# Autodesk Inventor assembly: BG301_trajan20_21
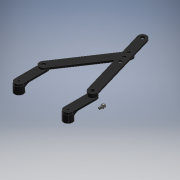
[picture p0: Inventor's stored thumbnail of the model, 180x180]
Saved by Autodesk Inventor 2022.2 (Build 262287000, 287)
## iProperties
Company: HTBLA Kaindorf
RuleStatus: InUse
Created: 2022-08-22
Part Number: BG301_trajan20_21
Project: Zeichenmaschine_v2
Material: Generisch
Description: gelenke
Document SubType Name: Assembly
Designer: trajan20
AfterDocNew0: iProperties-Editor_aufrufen
Author: jan
Keywords: 2021
## Documents named in this file (6)
- C:\Users\jan\Documents\DrawMachine\DrawMachineConstruction\Projekt\Zeichenmaschine_v2\BG301_trajan20_21_Zeichenmaschine_v2_gelenke.iam
- C:\Users\jan\Documents\DrawMachine\DrawMachineConstruction\Projekt\Zeichenmaschine_v2\BT301_trajan20_21_Zeichenmaschine_v2_gelenk 1.ipt
- C:\Users\jan\Documents\DrawMachine\DrawMachineConstruction\Projekt\Zeichenmaschine_v2\BT301_trajan20_21_Zeichenmaschine_v2_gelenk a.ipt
- C:\Users\jan\Documents\DrawMachine\DrawMachineConstruction\Projekt\Zeichenmaschine_v2\BT303_trajan20_21_Zeichenmaschine_v2_gelenk b.ipt
- C:\Users\jan\Documents\DrawMachine\DrawMachineConstruction\Projekt\Zeichenmaschine_v2\BT305_trajan20_21_Zeichenmaschine_v2_Platzhalter_steppermotor.ipt
- C:\Users\jan\Documents\DrawMachine\DrawMachineConstruction\Projekt\Zeichenmaschine_v2\Normteile\de-DE\ISO 4762(2)\ISO 4762 - M5 x 8ISO.ipt
## Components (7 placed, 5 different names)
1. BT301_trajan20_21_Zeichenmaschine_v2_gelenk 1:1 — Passend:1, Fluchtend:1, Winkel:1, Passend:9, Passend:15, Passend:16
2. BT301_trajan20_21_Zeichenmaschine_v2_gelenk a:1 — Passend:2, Passend:3, Passend:18
3. BT301_trajan20_21_Zeichenmaschine_v2_gelenk 1:2 — Passend:1, Fluchtend:1, Winkel:1, Passend:2, Passend:3, Passend:9, Passend:14, Passend:17
4. BT303_trajan20_21_Zeichenmaschine_v2_gelenk b:1 — Passend:18
5. BT305_trajan20_21_Zeichenmaschine_v2_Platzhalter_steppermotor:1 — Passend:14, Passend:17
6. BT305_trajan20_21_Zeichenmaschine_v2_Platzhalter_steppermotor:2 — Passend:15, Passend:16
7. ISO 4762 M5 x 8:1
## Relationships (11: Mate 9, Flush 1, Angle 1)
- Passend:1 [Mate] (120 mm): BT301_trajan20_21_Zeichenmaschine_v2_gelenk 1:1 ↔ BT301_trajan20_21_Zeichenmaschine_v2_gelenk 1:2
- Fluchtend:1 [Flush]: BT301_trajan20_21_Zeichenmaschine_v2_gelenk 1:1 ↔ BT301_trajan20_21_Zeichenmaschine_v2_gelenk 1:2
- Winkel:1 [Angle] (180 deg): BT301_trajan20_21_Zeichenmaschine_v2_gelenk 1:1 ↔ BT301_trajan20_21_Zeichenmaschine_v2_gelenk 1:2
- Passend:2 [Mate]: BT301_trajan20_21_Zeichenmaschine_v2_gelenk a:1 ↔ BT301_trajan20_21_Zeichenmaschine_v2_gelenk 1:2
- Passend:3 [Mate]: BT301_trajan20_21_Zeichenmaschine_v2_gelenk a:1 ↔ BT301_trajan20_21_Zeichenmaschine_v2_gelenk 1:2
- Passend:9 [Mate] (100 mm): BT301_trajan20_21_Zeichenmaschine_v2_gelenk 1:1 ↔ BT301_trajan20_21_Zeichenmaschine_v2_gelenk 1:2
- Passend:14 [Mate]: BT301_trajan20_21_Zeichenmaschine_v2_gelenk 1:2 ↔ BT305_trajan20_21_Zeichenmaschine_v2_Platzhalter_steppermotor:1
- Passend:15 [Mate]: BT301_trajan20_21_Zeichenmaschine_v2_gelenk 1:1 ↔ BT305_trajan20_21_Zeichenmaschine_v2_Platzhalter_steppermotor:2
- Passend:16 [Mate]: BT301_trajan20_21_Zeichenmaschine_v2_gelenk 1:1 ↔ BT305_trajan20_21_Zeichenmaschine_v2_Platzhalter_steppermotor:2
- Passend:17 [Mate]: BT301_trajan20_21_Zeichenmaschine_v2_gelenk 1:2 ↔ BT305_trajan20_21_Zeichenmaschine_v2_Platzhalter_steppermotor:1
- Passend:18 [Mate]: BT301_trajan20_21_Zeichenmaschine_v2_gelenk a:1 ↔ BT303_trajan20_21_Zeichenmaschine_v2_gelenk b:1
